# Autodesk Inventor assembly: MainAssembly
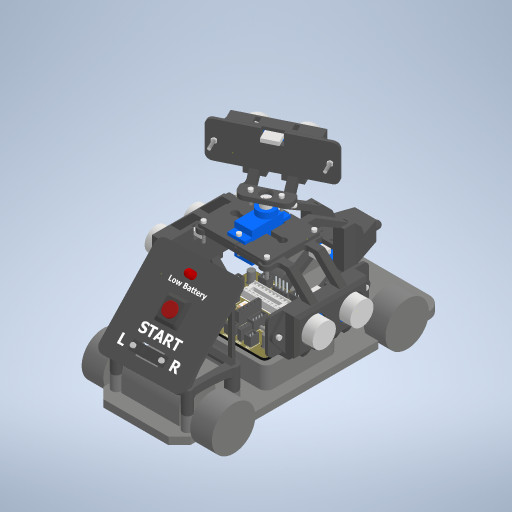
[picture p0: Inventor's stored thumbnail of the model, 512x512]
Saved by Autodesk Inventor 2024.2 (Build 282272000, 272)
## iProperties
Created: 2024-05-04
Part Number: MainAssembly
Document SubType Name: Assembly
Designer: ringl
Author: ringl
## Documents named in this file (26)
- C:\Users\ringl\OneDrive\Uni_PC_backup\Y4S2\EE579\Assignment\EE579-Skittles\CAD\Assembly\Main\MainAssembly.iam
- C:\Users\ringl\OneDrive\Uni_PC_backup\Y4S2\EE579\Assignment\EE579-Skittles\CAD\Components\CarApproximation02.ipt
- C:\Users\ringl\OneDrive\Uni_PC_backup\Y4S2\EE579\Assignment\EE579-Skittles\CAD\Bottom_Mount.ipt
- C:\Users\ringl\OneDrive\Uni_PC_backup\Y4S2\EE579\Assignment\EE579-Skittles\CAD\UltrasonicSensorMount02.ipt
- C:\Users\ringl\OneDrive\Uni_PC_backup\Y4S2\EE579\Assignment\EE579-Skittles\CAD\IRMount_bottom.ipt
- C:\Users\ringl\OneDrive\Uni_PC_backup\Y4S2\EE579\Assignment\EE579-Skittles\CAD\IRMount_top.ipt
- C:\Users\ringl\OneDrive\Uni_PC_backup\Y4S2\EE579\Assignment\EE579-Skittles\CAD\Top_Mount.ipt
- C:\Users\ringl\OneDrive\Uni_PC_backup\Y4S2\EE579\Assignment\EE579-Skittles\CAD\ServoFullMountInsert_left.ipt
- C:\Users\ringl\OneDrive\Uni_PC_backup\Y4S2\EE579\Assignment\EE579-Skittles\CAD\ServoFullMountInsert_right.ipt
- C:\Users\ringl\OneDrive\Uni_PC_backup\Y4S2\EE579\Assignment\EE579-Skittles\CAD\Components\UltrasonicSensor.ipt
- C:\Users\ringl\OneDrive\Uni_PC_backup\Y4S2\EE579\Assignment\EE579-Skittles\CAD\UltrasonicSensorMount_backplate03.ipt
- C:\Users\ringl\OneDrive\Uni_PC_backup\Y4S2\EE579\Assignment\EE579-Skittles\CAD\Components\M2x12.ipt
- C:\Users\ringl\OneDrive\Uni_PC_backup\Y4S2\EE579\Assignment\EE579-Skittles\CAD\Components\M2Nut.ipt
- C:\Users\ringl\OneDrive\Uni_PC_backup\Y4S2\EE579\Assignment\EE579-Skittles\CAD\ControlPanel_Bottom.ipt
- C:\Users\ringl\OneDrive\Uni_PC_backup\Y4S2\EE579\Assignment\EE579-Skittles\CAD\ControlPanel_Middle.ipt
- C:\Users\ringl\OneDrive\Uni_PC_backup\Y4S2\EE579\Assignment\EE579-Skittles\CAD\ControlPanel_Top.ipt
- C:\Users\ringl\OneDrive\Uni_PC_backup\Y4S2\EE579\Assignment\EE579-Skittles\CAD\PCB\EE579_Skittles_pcb\EE579_Skittles_pcb.iam
- C:\Users\ringl\OneDrive\Uni_PC_backup\Y4S2\EE579\Assignment\EE579-Skittles\CAD\Components\IR.ipt
- C:\Users\ringl\OneDrive\Uni_PC_backup\Y4S2\EE579\Assignment\EE579-Skittles\CAD\Components\SG-90-Servo.ipt
- C:\Users\ringl\OneDrive\Uni_PC_backup\Y4S2\EE579\Assignment\EE579-Skittles\CAD\Components\M2_Washer.ipt
- C:\Users\ringl\OneDrive\Uni_PC_backup\Y4S2\EE579\Assignment\EE579-Skittles\CAD\Components\ServoWings.ipt
- C:\Users\ringl\OneDrive\Uni_PC_backup\Y4S2\EE579\Assignment\EE579-Skittles\CAD\ServoUltrasonicMount.ipt
- C:\Users\ringl\OneDrive\Uni_PC_backup\Y4S2\EE579\Assignment\EE579-Skittles\CAD\Components\Red_LED.ipt
- C:\Users\ringl\OneDrive\Uni_PC_backup\Y4S2\EE579\Assignment\EE579-Skittles\CAD\Components\StartBtn.ipt
- C:\Users\ringl\OneDrive\Uni_PC_backup\Y4S2\EE579\Assignment\EE579-Skittles\CAD\Components\SlideSwitch.ipt
- C:\Users\ringl\OneDrive\Uni_PC_backup\Y4S2\EE579\Assignment\EE579-Skittles\CAD\Components\M2x8.ipt
## Components (65 placed, 25 different names)
1. CarApproximation02:1 — Mate:1, Mate:2, Mate:3, Mate:61, Mate:62, Mate:63, Mate:72, Mate:121, Mate:122, Mate:123, Mate:124
2. Bottom_Mount:1 — Mate:1, Mate:2, Mate:3, Mate:4, Mate:5, Mate:6, Mate:7, Mate:8, Mate:9, Mate:10, Mate:11, Mate:73, Mate:74
3. UltrasonicSensorMount02:1 — Mate:4, Mate:5, Mate:6, Mate:20, Mate:21, Mate:26, Mate:27, Mate:28, Mate:29, Mate:51, Mate:52
4. UltrasonicSensorMount02:2 — Mate:33, Mate:34, Mate:35, Mate:36, Mate:37, Mate:38, Mate:39, Mate:40, Mate:41, Mate:42, Mate:117, Mate:118, Mate:119
5. UltrasonicSensorMount02:3 — Mate:7, Mate:8, Mate:9, Mate:13, Mate:14, Mate:15, Mate:23, Mate:24, Mate:25, Mate:30, Mate:31, Mate:32, Mate:47, Mate:48, Mate:50
6. IRMount_bottom:1 — Mate:10, Mate:11, Mate:12, Flush:1, Flush:2, Mate:74, Mate:75, Mate:76
7. IRMount_top:1 — Mate:12, Flush:1, Flush:2
8. Top_Mount:1 — Mate:13, Mate:14, Mate:15, Mate:16, Mate:17, Mate:18, Mate:19, Mate:97, Mate:102, Mate:103, Mate:106, Mate:109
9. ServoFullMountInsert_left:1 — Mate:16, Mate:17, Mate:81, Mate:82, Mate:86, Mate:87
10. ServoFullMountInsert_right:1 — Mate:18, Mate:19, Mate:77, Mate:78, Mate:79, Mate:80, Mate:85, Mate:89, Mate:108, Mate:112
11. UltrasonicSensor:1 — Mate:20, Mate:21, Mate:26
12. UltrasonicSensor:2 — Mate:23, Mate:24, Mate:25
13. UltrasonicSensorMount_backplate03:1 — Mate:30, Mate:31, Mate:32, Mate:49, Mate:59, Mate:60
14. UltrasonicSensorMount_backplate03:2 — Mate:27, Mate:28, Mate:29, Mate:55, Mate:56
15. UltrasonicSensorMount_backplate03:3 — Mate:36, Mate:37, Mate:38, Mate:45, Mate:46
16. M2x12:1 — Mate:52, Mate:53
17. M2x12:2 — Mate:51, Mate:54
18. M2x12:3 — Mate:49, Mate:50, Mate:58
19. M2x12:4 — Mate:47, Mate:48, Mate:57
20. M2x12:5 — Mate:40, Mate:41, Mate:43
21. M2x12:6 — Mate:39, Mate:42, Mate:44
22. UltrasonicSensor:3 — Mate:33, Mate:34, Mate:35
23. M2Nut:1 — Mate:44, Mate:45
24. M2Nut:2 — Mate:43, Mate:46
25. M2Nut:3 — Mate:53, Mate:56
26. M2Nut:4 — Mate:54, Mate:55
27. M2Nut:5 — Mate:57, Mate:59
28. M2Nut:6 — Mate:58, Mate:60
29. ControlPanel_Bottom:1 — Mate:61, Mate:62, Mate:63, Mate:64, Mate:65, Mate:66, Mate:67, Mate:68, Mate:69
30. ControlPanel_Middle:1 — Mate:64, Mate:65, Mate:69, Tangent:1
31. ControlPanel_Middle:2 — Mate:66, Mate:67, Mate:68, Mate:70, Mate:71
32. ControlPanel_Top:1 — Mate:70, Mate:71, Tangent:1, Mate:120, Flush:3, Mate:125, Mate:126, Mate:127, Mate:128, Mate:129, Mate:136, Mate:137
33. EE579_Skittles_pcb:1 [sub-assembly] — Mate:72, Mate:73
34. IR:1 — Mate:75, Mate:76
35. SG-90-Servo:1 — Mate:77, Mate:78, Mate:83, Mate:84, Mate:88, Mate:90, Mate:111, Mate:112, Mate:113
36. M2x12:7 — Mate:80, Mate:89, Mate:94, Mate:100
37. M2x12:8 — Mate:82, Mate:87, Mate:95, Mate:98
38. M2x12:9 — Mate:79, Mate:85, Mate:91, Mate:101
39. M2x12:10 — Mate:81, Mate:86, Mate:92, Mate:99
40. M2x12:11 — Mate:84, Mate:88, Mate:96
41. M2x12:12 — Mate:83, Mate:90, Mate:93
42. M2Nut:7 — Mate:93, Mate:108
43. M2Nut:8 — Mate:96, Mate:97
44. M2Nut:9 — Mate:91, Mate:104
45. M2Nut:10 — Mate:94, Mate:105
46. M2Nut:11 — Mate:95, Mate:107
47. M2Nut:12 — Mate:92, Mate:110
48. M2_Washer:1 — Mate:98, Mate:106, Mate:107
49. M2_Washer:2 — Mate:99, Mate:109, Mate:110
50. M2_Washer:3 — Mate:100, Mate:102, Mate:105
51. M2_Washer:4 — Mate:101, Mate:103, Mate:104
52. ServoWings:1 — Mate:111, Mate:113, Mate:114, Mate:115, Mate:116, Mate:138, Mate:139
53. ServoUltrasonicMount:1 — Mate:114, Mate:115, Mate:116, Mate:117, Mate:118, Mate:119, Mate:140, Mate:141, Mate:142, Mate:143
54. Red_LED:1 — Mate:120, Flush:3
55. M2x12:13 — Mate:121, Mate:124
56. M2x12:14 — Mate:122, Mate:123
57. StartBtn:1 — Mate:125, Mate:126
58. SlideSwitch:2 — Mate:127, Mate:128, Mate:129, Mate:130, Mate:131, Mate:132, Mate:133
59. M2x8:1 — Mate:131, Mate:132, Mate:135
60. M2x8:2 — Mate:130, Mate:133, Mate:134
61. M2Nut:13 — Mate:134, Mate:136
62. M2Nut:14 — Mate:135, Mate:137
63. M2x8:3 — Mate:138, Mate:139
64. M2x8:4 — Mate:140, Mate:143
65. M2x8:5 — Mate:141, Mate:142
## Relationships (146: Mate 142, Flush 3, Tangent 1)
- Mate:1: CarApproximation02:1 ↔ Bottom_Mount:1
- Mate:2: CarApproximation02:1 ↔ Bottom_Mount:1
- Mate:3: CarApproximation02:1 ↔ Bottom_Mount:1
- Mate:4: Bottom_Mount:1 ↔ UltrasonicSensorMount02:1
- Mate:5 (0.1 mm): Bottom_Mount:1 ↔ UltrasonicSensorMount02:1
- Mate:6 (0.1 mm): Bottom_Mount:1 ↔ UltrasonicSensorMount02:1
- Mate:7: Bottom_Mount:1 ↔ UltrasonicSensorMount02:3
- Mate:8 (0.1 mm): Bottom_Mount:1 ↔ UltrasonicSensorMount02:3
- Mate:9 (0.1 mm): Bottom_Mount:1 ↔ UltrasonicSensorMount02:3
- Mate:10: Bottom_Mount:1 ↔ IRMount_bottom:1
- Mate:11 (0.1 mm): Bottom_Mount:1 ↔ IRMount_bottom:1
- Mate:12: IRMount_bottom:1 ↔ IRMount_top:1
- Flush:1: IRMount_bottom:1 ↔ IRMount_top:1
- Flush:2: IRMount_bottom:1 ↔ IRMount_top:1
- Mate:13: UltrasonicSensorMount02:3 ↔ Top_Mount:1
- Mate:14 (0.1 mm): UltrasonicSensorMount02:3 ↔ Top_Mount:1
- Mate:15 (0.1 mm): UltrasonicSensorMount02:3 ↔ Top_Mount:1
- Mate:16: Top_Mount:1 ↔ ServoFullMountInsert_left:1
- Mate:17: Top_Mount:1 ↔ ServoFullMountInsert_left:1
- Mate:18: Top_Mount:1 ↔ ServoFullMountInsert_right:1
- Mate:19: Top_Mount:1 ↔ ServoFullMountInsert_right:1
- Mate:20: UltrasonicSensorMount02:1 ↔ UltrasonicSensor:1
- Mate:21: UltrasonicSensorMount02:1 ↔ UltrasonicSensor:1
- Mate:23: UltrasonicSensorMount02:3 ↔ UltrasonicSensor:2
- Mate:24: UltrasonicSensorMount02:3 ↔ UltrasonicSensor:2
- Mate:25: UltrasonicSensorMount02:3 ↔ UltrasonicSensor:2
- Mate:26: UltrasonicSensorMount02:1 ↔ UltrasonicSensor:1
- Mate:27: UltrasonicSensorMount02:1 ↔ UltrasonicSensorMount_backplate03:2
- Mate:28: UltrasonicSensorMount02:1 ↔ UltrasonicSensorMount_backplate03:2
- Mate:29: UltrasonicSensorMount02:1 ↔ UltrasonicSensorMount_backplate03:2
- Mate:30: UltrasonicSensorMount02:3 ↔ UltrasonicSensorMount_backplate03:1
- Mate:31: UltrasonicSensorMount02:3 ↔ UltrasonicSensorMount_backplate03:1
- Mate:32: UltrasonicSensorMount02:3 ↔ UltrasonicSensorMount_backplate03:1
- Mate:33: UltrasonicSensorMount02:2 ↔ UltrasonicSensor:3
- Mate:34: UltrasonicSensorMount02:2 ↔ UltrasonicSensor:3
- Mate:35: UltrasonicSensorMount02:2 ↔ UltrasonicSensor:3
- Mate:36: UltrasonicSensorMount02:2 ↔ UltrasonicSensorMount_backplate03:3
- Mate:37: UltrasonicSensorMount02:2 ↔ UltrasonicSensorMount_backplate03:3
- Mate:38: UltrasonicSensorMount02:2 ↔ UltrasonicSensorMount_backplate03:3
- Mate:39: UltrasonicSensorMount02:2 ↔ M2x12:6
- Mate:40: UltrasonicSensorMount02:2 ↔ M2x12:5
- Mate:41: UltrasonicSensorMount02:2 ↔ M2x12:5
- Mate:42: UltrasonicSensorMount02:2 ↔ M2x12:6
- Mate:43: M2x12:5 ↔ M2Nut:2
- Mate:44: M2x12:6 ↔ M2Nut:1
- Mate:45: UltrasonicSensorMount_backplate03:3 ↔ M2Nut:1
- Mate:46: UltrasonicSensorMount_backplate03:3 ↔ M2Nut:2
- Mate:47: UltrasonicSensorMount02:3 ↔ M2x12:4
- Mate:48: UltrasonicSensorMount02:3 ↔ M2x12:4
- Mate:49: UltrasonicSensorMount_backplate03:1 ↔ M2x12:3
- Mate:50: UltrasonicSensorMount02:3 ↔ M2x12:3
- Mate:51: UltrasonicSensorMount02:1 ↔ M2x12:2
- Mate:52: UltrasonicSensorMount02:1 ↔ M2x12:1
- Mate:53: M2x12:1 ↔ M2Nut:3
- Mate:54: M2x12:2 ↔ M2Nut:4
- Mate:55: UltrasonicSensorMount_backplate03:2 ↔ M2Nut:4
- Mate:56: UltrasonicSensorMount_backplate03:2 ↔ M2Nut:3
- Mate:57: M2x12:4 ↔ M2Nut:5
- Mate:58: M2x12:3 ↔ M2Nut:6
- Mate:59: UltrasonicSensorMount_backplate03:1 ↔ M2Nut:5
- Mate:60: UltrasonicSensorMount_backplate03:1 ↔ M2Nut:6
- Mate:61: CarApproximation02:1 ↔ ControlPanel_Bottom:1
- Mate:62: CarApproximation02:1 ↔ ControlPanel_Bottom:1
- Mate:63: CarApproximation02:1 ↔ ControlPanel_Bottom:1
- Mate:64: ControlPanel_Bottom:1 ↔ ControlPanel_Middle:1
- Mate:65: ControlPanel_Bottom:1 ↔ ControlPanel_Middle:1
- Mate:66: ControlPanel_Bottom:1 ↔ ControlPanel_Middle:2
- Mate:67: ControlPanel_Bottom:1 ↔ ControlPanel_Middle:2
- Mate:68: ControlPanel_Bottom:1 ↔ ControlPanel_Middle:2
- Mate:69: ControlPanel_Bottom:1 ↔ ControlPanel_Middle:1
- Mate:70: ControlPanel_Middle:2 ↔ ControlPanel_Top:1
- Mate:71 (3 mm): ControlPanel_Middle:2 ↔ ControlPanel_Top:1
- Tangent:1 (7 mm): ControlPanel_Middle:1 ↔ ControlPanel_Top:1
- Mate:72: CarApproximation02:1 ↔ EE579_Skittles_pcb:1
- Mate:73: Bottom_Mount:1 ↔ EE579_Skittles_pcb:1
- Mate:74 (0.1 mm): Bottom_Mount:1 ↔ IRMount_bottom:1
- Mate:75: IRMount_bottom:1 ↔ IR:1
- Mate:76: IRMount_bottom:1 ↔ IR:1
- Mate:77: ServoFullMountInsert_right:1 ↔ SG-90-Servo:1
- Mate:78 (0.8 mm): ServoFullMountInsert_right:1 ↔ SG-90-Servo:1
- Mate:79: ServoFullMountInsert_right:1 ↔ M2x12:9
- Mate:80: ServoFullMountInsert_right:1 ↔ M2x12:7
- Mate:81: ServoFullMountInsert_left:1 ↔ M2x12:10
- Mate:82: ServoFullMountInsert_left:1 ↔ M2x12:8
- Mate:83: SG-90-Servo:1 ↔ M2x12:12
- Mate:84: SG-90-Servo:1 ↔ M2x12:11
- Mate:85: ServoFullMountInsert_right:1 ↔ M2x12:9
- Mate:86: ServoFullMountInsert_left:1 ↔ M2x12:10
- Mate:87: ServoFullMountInsert_left:1 ↔ M2x12:8
- Mate:88: SG-90-Servo:1 ↔ M2x12:11
- Mate:89: ServoFullMountInsert_right:1 ↔ M2x12:7
- Mate:90: SG-90-Servo:1 ↔ M2x12:12
- Mate:91: M2x12:9 ↔ M2Nut:9
- Mate:92: M2x12:10 ↔ M2Nut:12
- Mate:93: M2x12:12 ↔ M2Nut:7
- Mate:94: M2x12:7 ↔ M2Nut:10
- Mate:95: M2x12:8 ↔ M2Nut:11
- Mate:96: M2x12:11 ↔ M2Nut:8
- Mate:97: Top_Mount:1 ↔ M2Nut:8
- Mate:98: M2x12:8 ↔ M2_Washer:1
- Mate:99: M2x12:10 ↔ M2_Washer:2
- Mate:100: M2x12:7 ↔ M2_Washer:3
- Mate:101: M2x12:9 ↔ M2_Washer:4
- Mate:102: Top_Mount:1 ↔ M2_Washer:3
- Mate:103: Top_Mount:1 ↔ M2_Washer:4
- Mate:104: M2Nut:9 ↔ M2_Washer:4
- Mate:105: M2Nut:10 ↔ M2_Washer:3
- Mate:106: Top_Mount:1 ↔ M2_Washer:1
- Mate:107: M2Nut:11 ↔ M2_Washer:1
- Mate:108: ServoFullMountInsert_right:1 ↔ M2Nut:7
- Mate:109: Top_Mount:1 ↔ M2_Washer:2
- Mate:110: M2Nut:12 ↔ M2_Washer:2
- Mate:111: SG-90-Servo:1 ↔ ServoWings:1
- Mate:112 (0.5 mm): ServoFullMountInsert_right:1 ↔ SG-90-Servo:1
- Mate:113: SG-90-Servo:1 ↔ ServoWings:1
- Mate:114: ServoWings:1 ↔ ServoUltrasonicMount:1
- Mate:115: ServoWings:1 ↔ ServoUltrasonicMount:1
- Mate:116: ServoWings:1 ↔ ServoUltrasonicMount:1
- Mate:117: UltrasonicSensorMount02:2 ↔ ServoUltrasonicMount:1
- Mate:118 (0.1 mm): UltrasonicSensorMount02:2 ↔ ServoUltrasonicMount:1
- Mate:119 (0.1 mm): UltrasonicSensorMount02:2 ↔ ServoUltrasonicMount:1
- Mate:120: ControlPanel_Top:1 ↔ Red_LED:1
- Flush:3: ControlPanel_Top:1 ↔ Red_LED:1
- Mate:121: CarApproximation02:1 ↔ M2x12:13
- Mate:122: CarApproximation02:1 ↔ M2x12:14
- Mate:123: CarApproximation02:1 ↔ M2x12:14
- Mate:124: CarApproximation02:1 ↔ M2x12:13
- Mate:125: ControlPanel_Top:1 ↔ StartBtn:1
- Mate:126: ControlPanel_Top:1 ↔ StartBtn:1
- Mate:127: ControlPanel_Top:1 ↔ SlideSwitch:2
- Mate:128: ControlPanel_Top:1 ↔ SlideSwitch:2
- Mate:129: ControlPanel_Top:1 ↔ SlideSwitch:2
- Mate:130: SlideSwitch:2 ↔ M2x8:2
- Mate:131: SlideSwitch:2 ↔ M2x8:1
- Mate:132: SlideSwitch:2 ↔ M2x8:1
- Mate:133: SlideSwitch:2 ↔ M2x8:2
- Mate:134: M2x8:2 ↔ M2Nut:13
- Mate:135: M2x8:1 ↔ M2Nut:14
- Mate:136: ControlPanel_Top:1 ↔ M2Nut:13
- Mate:137: ControlPanel_Top:1 ↔ M2Nut:14
- Mate:138: ServoWings:1 ↔ M2x8:3
- Mate:139: ServoWings:1 ↔ M2x8:3
- Mate:140: ServoUltrasonicMount:1 ↔ M2x8:4
- Mate:141: ServoUltrasonicMount:1 ↔ M2x8:5
- Mate:142: ServoUltrasonicMount:1 ↔ M2x8:5
- Mate:143: ServoUltrasonicMount:1 ↔ M2x8:4
